# Autodesk Inventor assembly: Print
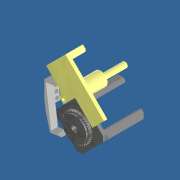
[picture p0: Inventor's stored thumbnail of the model, 180x180]
Saved by Autodesk Inventor 2020 (Build 240168000, 168)
## iProperties
Created: 2019-12-16
Part Number: Print
Document SubType Name: Assembly
Designer: Jack
Author: Jack
## Documents named in this file (4)
- D:\Code\Python\EV3_Cuber\3D Model\Print.iam
- D:\Code\Python\EV3_Cuber\3D Model\HolderGear.ipt
- D:\Code\Python\EV3_Cuber\3D Model\Hand.ipt
- D:\Code\Python\EV3_Cuber\3D Model\HolderShaft.ipt
## Components (3 placed, 3 different names)
1. Hand:1 — Flush:1, Mate:3, Mate:4
2. HolderGear:1 — Flush:1, Flush:2, Angle:2, Mate:2, Mate:3, Mate:4
3. HolderShaft:1 — Flush:2, Angle:2, Mate:2
## Relationships (6: Mate 3, Flush 2, Angle 1)
- Flush:1: Hand:1 ↔ HolderGear:1
- Flush:2: HolderGear:1 ↔ HolderShaft:1
- Angle:2 (0 deg): HolderGear:1 ↔ HolderShaft:1
- Mate:2 (-98.5 mm): HolderGear:1 ↔ HolderShaft:1
- Mate:3 (14 mm): Hand:1 ↔ HolderGear:1
- Mate:4 (19 mm): Hand:1 ↔ HolderGear:1
